# Autodesk Inventor assembly: Ensamble_cuerpo
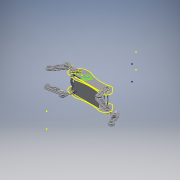
[picture p0: Inventor's stored thumbnail of the model, 180x180]
Saved by Autodesk Inventor 2019 (Build 230136000, 136)
## iProperties
Created: 2020-02-15
Part Number: Ensamble_cuerpo
Material: Genérico
Document SubType Name: Assembly
Designer: Mafer1
Author: Mafer1
## Documents named in this file (6)
- E:\Escritorio\Temporal\Documentos\Robótica I\ProyectoCuadrupedo\Proyecto1\Proyecto1\Ensamble_cuerpo.iam
- E:\Escritorio\Temporal\Documentos\Robótica I\ProyectoCuadrupedo\Proyecto1\Proyecto1\Cuerpo - Lateral.ipt
- E:\Escritorio\Temporal\Documentos\Robótica I\ProyectoCuadrupedo\Proyecto1\Proyecto1\Cuerpo - Base.ipt
- E:\Escritorio\Temporal\Documentos\Robótica I\ProyectoCuadrupedo\Proyecto1\Proyecto1\Cuerpo - Unión Laterales.ipt
- E:\Escritorio\Temporal\Documentos\Robótica I\ProyectoCuadrupedo\Proyecto1\Proyecto1\Ensamble_Pierna.iam
- E:\Escritorio\Temporal\Documentos\Robótica I\ProyectoCuadrupedo\Proyecto1\Proyecto1\Ensamble_Pierna_delantera.iam
## Components (11 placed, 5 different names)
1. lateral1:2 — Coincidencia:1, Coincidencia:2, Coincidencia:3, Coincidencia:28, Coincidencia:29, Coincidencia:30, Coincidencia:31, Coincidencia:32, Coincidencia:33
2. base:1 — Coincidencia:1, Coincidencia:2, Coincidencia:3, Coincidencia:4, Coincidencia:5, Coincidencia:6
3. lateral1:3 — Coincidencia:4, Coincidencia:5, Coincidencia:6, Coincidencia:7, Coincidencia:8, Coincidencia:9, Coincidencia:10, Coincidencia:11, Coincidencia:12, Coincidencia:13, Coincidencia:14, Coincidencia:15, Coincidencia:16, Coincidencia:17, Coincidencia:18, Coincidencia:22, Coincidencia:23, Coincidencia:24, Coincidencia:25, Coincidencia:26, Coincidencia:27
4. union_lateral:1 — Coincidencia:7, Coincidencia:8, Coincidencia:9
5. union_lateral:2 — Coincidencia:10, Coincidencia:11, Coincidencia:12
6. union_lateral:3 — Coincidencia:13, Coincidencia:14, Coincidencia:15
7. union_lateral:4 — Coincidencia:16, Coincidencia:17, Coincidencia:18
8. Ensamble_Pierna:2 [sub-assembly] — Coincidencia:22, Coincidencia:23, Coincidencia:24
9. Ensamble_Pierna_delantera:1 [sub-assembly] — Coincidencia:25, Coincidencia:26, Coincidencia:27
10. Ensamble_Pierna_delantera:3 [sub-assembly] — Coincidencia:28, Coincidencia:29, Coincidencia:30
11. Ensamble_Pierna:3 [sub-assembly] — Coincidencia:31, Coincidencia:32, Coincidencia:33
## Relationships (30: Mate 30)
- Coincidencia:1 [Mate] (-3.3 mm): lateral1:2 ↔ base:1
- Coincidencia:2 [Mate]: lateral1:2 ↔ base:1
- Coincidencia:3 [Mate]: lateral1:2 ↔ base:1
- Coincidencia:4 [Mate] (-3.3 mm): base:1 ↔ lateral1:3
- Coincidencia:5 [Mate]: base:1 ↔ lateral1:3
- Coincidencia:6 [Mate]: base:1 ↔ lateral1:3
- Coincidencia:7 [Mate]: lateral1:3 ↔ union_lateral:1
- Coincidencia:8 [Mate]: lateral1:3 ↔ union_lateral:1
- Coincidencia:9 [Mate]: lateral1:3 ↔ union_lateral:1
- Coincidencia:10 [Mate]: lateral1:3 ↔ union_lateral:2
- Coincidencia:11 [Mate]: lateral1:3 ↔ union_lateral:2
- Coincidencia:12 [Mate]: lateral1:3 ↔ union_lateral:2
- Coincidencia:13 [Mate]: lateral1:3 ↔ union_lateral:3
- Coincidencia:14 [Mate]: lateral1:3 ↔ union_lateral:3
- Coincidencia:15 [Mate]: lateral1:3 ↔ union_lateral:3
- Coincidencia:16 [Mate]: lateral1:3 ↔ union_lateral:4
- Coincidencia:17 [Mate]: lateral1:3 ↔ union_lateral:4
- Coincidencia:18 [Mate]: lateral1:3 ↔ union_lateral:4
- Coincidencia:22 [Mate]: lateral1:3 ↔ Ensamble_Pierna:2
- Coincidencia:23 [Mate]: lateral1:3 ↔ Ensamble_Pierna:2
- Coincidencia:24 [Mate]: lateral1:3 ↔ Ensamble_Pierna:2
- Coincidencia:25 [Mate]: lateral1:3 ↔ Ensamble_Pierna_delantera:1
- Coincidencia:26 [Mate]: lateral1:3 ↔ Ensamble_Pierna_delantera:1
- Coincidencia:27 [Mate]: lateral1:3 ↔ Ensamble_Pierna_delantera:1
- Coincidencia:28 [Mate]: lateral1:2 ↔ Ensamble_Pierna_delantera:3
- Coincidencia:29 [Mate]: lateral1:2 ↔ Ensamble_Pierna_delantera:3
- Coincidencia:30 [Mate]: lateral1:2 ↔ Ensamble_Pierna_delantera:3
- Coincidencia:31 [Mate]: lateral1:2 ↔ Ensamble_Pierna:3
- Coincidencia:32 [Mate]: lateral1:2 ↔ Ensamble_Pierna:3
- Coincidencia:33 [Mate]: lateral1:2 ↔ Ensamble_Pierna:3
